# Autodesk Inventor assembly: 조립품1
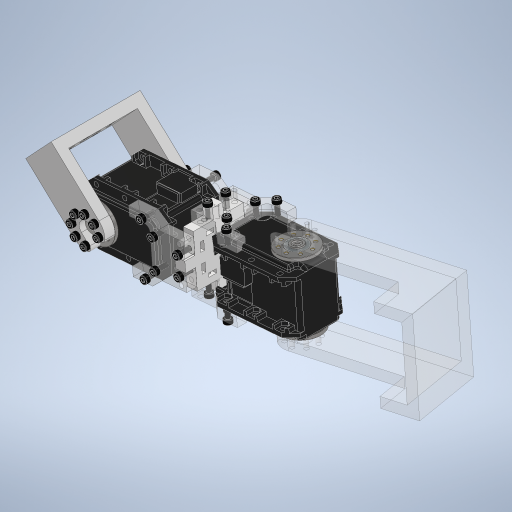
[picture p0: Inventor's stored thumbnail of the model, 512x512]
Saved by Autodesk Inventor 2024 (Build 280153000, 153)
## iProperties
Created: 2024-09-18
Part Number: 조립품1
Document SubType Name: Assembly
Designer: Eungang
Author: Eungang
## Documents named in this file (10)
- C:\Users\Eungang\Documents\Inventor\FIGHTING_ROBOT_FINAL\부품\Arm_Right\Right_Arm.iam
- C:\Users\Eungang\Documents\Inventor\FIGHTING_ROBOT_FINAL\부품\다이나믹셀\MX-28T_R.ipt
- C:\Users\Eungang\Documents\Inventor\FIGHTING_ROBOT_FINAL\부품\아이들러\28아이들러.iam
- C:\Users\Eungang\Documents\Inventor\FIGHTING_ROBOT_FINAL\부품\혼\28Horn.ipt
- C:\Users\Eungang\Documents\Inventor\FIGHTING_ROBOT_FINAL\부품\Bolt_Washer_Nut\CSH-ST-M2_5-8_203.ipt
- C:\Users\Eungang\Documents\Inventor\FIGHTING_ROBOT_FINAL\부품\Bolt_Washer_Nut\Arm_bolt_set_2_5_8 x 6.iam
- C:\Users\Eungang\Documents\Inventor\FIGHTING_ROBOT_FINAL\부품\Bolt_Washer_Nut\arm_motor_connect.ipt
- C:\Users\Eungang\Documents\Inventor\FIGHTING_ROBOT_FINAL\부품\Arm_Right\arm_motor_connecter_bridge.ipt
- C:\Users\Eungang\Documents\Inventor\FIGHTING_ROBOT_FINAL\부품\Arm_Right\hand.ipt
- C:\Users\Eungang\Documents\Inventor\FIGHTING_ROBOT_FINAL\부품\Arm_Right\arm_connect_3.ipt
## Components (30 placed, 8 different names)
1. MX-28T_R:1 — 삽입:1, 삽입:2, 삽입:47, 삽입:48, 삽입:49, 삽입:50
2. 28아이들러:1 [sub-assembly] — 삽입:2
3. 28Horn:1 — 삽입:1, 삽입:62
4. Arm_bolt_set_2_5_8 x 6:1 [sub-assembly] — 삽입:58, 삽입:59
5. Arm_bolt_set_2_5_8 x 6:2 [sub-assembly] — 삽입:51, 삽입:52
6. Arm_bolt_set_2_5_8 x 6:3 [sub-assembly] — 삽입:77, 삽입:78
7. Arm_bolt_set_2_5_8 x 6:4 [sub-assembly] — 삽입:80, 삽입:84, 삽입:85, 삽입:86
8. arm_motor_connecter_bridge:1 — 메이트:2, 삽입:55, 삽입:85, 삽입:86, 메이트:3, 삽입:87
9. arm_connect_3:1 — 삽입:62, 삽입:63, 삽입:64, 삽입:65, 삽입:66, 삽입:67, 삽입:68, 삽입:69, 삽입:70, 삽입:71, 삽입:72, 삽입:73, 삽입:74, 삽입:75, 삽입:76
10. arm_motor_connecter_bridge:2 — 삽입:49, 삽입:50, 삽입:51, 삽입:52, 삽입:55, 삽입:87
11. arm_motor_connecter_bridge:3 — 삽입:47, 삽입:48, 삽입:58, 삽입:59
12. arm_motor_connecter_bridge:5 — 메이트:2, 삽입:77, 삽입:78, 메이트:3
13. CSH-ST-M2_5-8_203:1 — 삽입:63
14. CSH-ST-M2_5-8_203:2 — 삽입:64
15. CSH-ST-M2_5-8_203:3 — 삽입:65
16. CSH-ST-M2_5-8_203:4 — 삽입:66
17. CSH-ST-M2_5-8_203:5 — 삽입:68
18. CSH-ST-M2_5-8_203:6 — 삽입:67
19. CSH-ST-M2_5-8_203:7 — 삽입:69
20. CSH-ST-M2_5-8_203:8 — 삽입:70
21. CSH-ST-M2_5-8_203:9 — 삽입:71
22. CSH-ST-M2_5-8_203:10 — 삽입:72
23. CSH-ST-M2_5-8_203:11 — 삽입:73
24. CSH-ST-M2_5-8_203:12 — 삽입:74
25. CSH-ST-M2_5-8_203:13 — 삽입:75
26. CSH-ST-M2_5-8_203:14 — 삽입:76
27. MX-28T_R:2 — 삽입:80, 삽입:81, 삽입:82, 삽입:84
28. 28아이들러:2 [sub-assembly] — 삽입:82
29. hand:1 — 삽입:83
30. 28Horn:2 — 삽입:81, 삽입:83
## Relationships (38: Insert 36, Mate 2)
- 삽입:1 [Insert] (0.75 mm): MX-28T_R:1 ↔ 28Horn:1
- 삽입:2 [Insert] (0.75 mm): MX-28T_R:1 ↔ 28아이들러:1
- 삽입:47 [Insert]: MX-28T_R:1 ↔ arm_motor_connecter_bridge:3
- 삽입:48 [Insert]: MX-28T_R:1 ↔ arm_motor_connecter_bridge:3
- 삽입:49 [Insert]: MX-28T_R:1 ↔ arm_motor_connecter_bridge:2
- 삽입:50 [Insert]: MX-28T_R:1 ↔ arm_motor_connecter_bridge:2
- 삽입:51 [Insert]: Arm_bolt_set_2_5_8 x 6:2 ↔ arm_motor_connecter_bridge:2
- 삽입:52 [Insert]: Arm_bolt_set_2_5_8 x 6:2 ↔ arm_motor_connecter_bridge:2
- 메이트:2 [Mate] (0.1 mm): arm_motor_connecter_bridge:1 ↔ arm_motor_connecter_bridge:5
- 삽입:55 [Insert] (0.1 mm): arm_motor_connecter_bridge:1 ↔ arm_motor_connecter_bridge:2
- 삽입:58 [Insert]: Arm_bolt_set_2_5_8 x 6:1 ↔ arm_motor_connecter_bridge:3
- 삽입:59 [Insert]: Arm_bolt_set_2_5_8 x 6:1 ↔ arm_motor_connecter_bridge:3
- 삽입:62 [Insert] (0.1 mm): 28Horn:1 ↔ arm_connect_3:1
- 삽입:63 [Insert]: arm_connect_3:1 ↔ CSH-ST-M2_5-8_203:1
- 삽입:64 [Insert]: arm_connect_3:1 ↔ CSH-ST-M2_5-8_203:2
- 삽입:65 [Insert]: arm_connect_3:1 ↔ CSH-ST-M2_5-8_203:3
- 삽입:66 [Insert]: arm_connect_3:1 ↔ CSH-ST-M2_5-8_203:4
- 삽입:67 [Insert]: arm_connect_3:1 ↔ CSH-ST-M2_5-8_203:6
- 삽입:68 [Insert]: arm_connect_3:1 ↔ CSH-ST-M2_5-8_203:5
- 삽입:69 [Insert]: arm_connect_3:1 ↔ CSH-ST-M2_5-8_203:7
- 삽입:70 [Insert]: arm_connect_3:1 ↔ CSH-ST-M2_5-8_203:8
- 삽입:71 [Insert]: arm_connect_3:1 ↔ CSH-ST-M2_5-8_203:9
- 삽입:72 [Insert]: arm_connect_3:1 ↔ CSH-ST-M2_5-8_203:10
- 삽입:73 [Insert]: arm_connect_3:1 ↔ CSH-ST-M2_5-8_203:11
- 삽입:74 [Insert]: arm_connect_3:1 ↔ CSH-ST-M2_5-8_203:12
- 삽입:75 [Insert]: arm_connect_3:1 ↔ CSH-ST-M2_5-8_203:13
- 삽입:76 [Insert]: arm_connect_3:1 ↔ CSH-ST-M2_5-8_203:14
- 삽입:77 [Insert]: Arm_bolt_set_2_5_8 x 6:3 ↔ arm_motor_connecter_bridge:5
- 삽입:78 [Insert]: Arm_bolt_set_2_5_8 x 6:3 ↔ arm_motor_connecter_bridge:5
- 삽입:80 [Insert]: Arm_bolt_set_2_5_8 x 6:4 ↔ MX-28T_R:2
- 삽입:81 [Insert] (0.75 mm): MX-28T_R:2 ↔ 28Horn:2
- 삽입:82 [Insert] (0.75 mm): MX-28T_R:2 ↔ 28아이들러:2
- 삽입:83 [Insert] (0.1 mm): hand:1 ↔ 28Horn:2
- 삽입:84 [Insert]: Arm_bolt_set_2_5_8 x 6:4 ↔ MX-28T_R:2
- 삽입:85 [Insert]: Arm_bolt_set_2_5_8 x 6:4 ↔ arm_motor_connecter_bridge:1
- 삽입:86 [Insert]: Arm_bolt_set_2_5_8 x 6:4 ↔ arm_motor_connecter_bridge:1
- 메이트:3 [Mate] (0.1 mm): arm_motor_connecter_bridge:1 ↔ arm_motor_connecter_bridge:5
- 삽입:87 [Insert] (0.1 mm): arm_motor_connecter_bridge:1 ↔ arm_motor_connecter_bridge:2
